# Autodesk Inventor assembly: RoboMuse_Docked
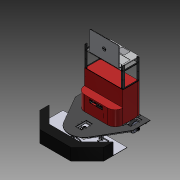
[picture p0: Inventor's stored thumbnail of the model, 180x180]
Saved by Autodesk Inventor 2018 (Build 220112000, 112)
## iProperties
Created: 2017-06-02
Part Number: RoboMuse_Docked
Document SubType Name: Assembly
Designer: AYUSH SHUKLA
Author: AYUSH SHUKLA
## Documents named in this file (6)
- C:\Study\BTP2\Robomuse Inventor CAD\RoboMuse_Docked.iam
- C:\Study\BTP2\Robomuse Inventor CAD\Robomuse.iam
- C:\Study\BTP2\Robomuse Inventor CAD\Dock.iam
- C:\Study\BTP2\Robomuse Inventor CAD\terminal.iam
- C:\Study\BTP2\Robomuse Inventor CAD\terminal_MIR.iam
- C:\Study\BTP2\Robomuse Inventor CAD\terminal_front.iam
## Components (5 placed, 5 different names)
1. Dock:1 [sub-assembly] — Mate:1, Angle:1, Angle:2, Flush:1, Flush:2
2. Robomuse:1 [sub-assembly] — Mate:1, Angle:1, Angle:2, Mate:2, Flush:2, Mate:3, Mate:4, Mate:5, Mate:6, Mate:7, Angle:3
3. terminal:1 [sub-assembly] — Mate:3, Mate:4
4. terminal_MIR:1 [sub-assembly] — Mate:5, Mate:6
5. terminal_front:1 [sub-assembly] — Mate:7, Angle:3, Flush:3
## Relationships (13: Mate 7, Angle 3, Flush 3)
- Mate:1 (-63.5 mm): Dock:1 ↔ Robomuse:1
- Angle:1 (0 deg): Dock:1 ↔ Robomuse:1
- Angle:2 (0 deg): Dock:1 ↔ Robomuse:1
- Flush:1 (50 mm): Dock:1
- Mate:2: Robomuse:1
- Flush:2: Dock:1 ↔ Robomuse:1
- Mate:3: Robomuse:1 ↔ terminal:1
- Mate:4: Robomuse:1 ↔ terminal:1
- Mate:5: Robomuse:1 ↔ terminal_MIR:1
- Mate:6: Robomuse:1 ↔ terminal_MIR:1
- Mate:7: Robomuse:1 ↔ terminal_front:1
- Angle:3 (0 deg): Robomuse:1 ↔ terminal_front:1
- Flush:3 (-12.7 mm): terminal_front:1
